# Autodesk Inventor assembly: клешня сбора
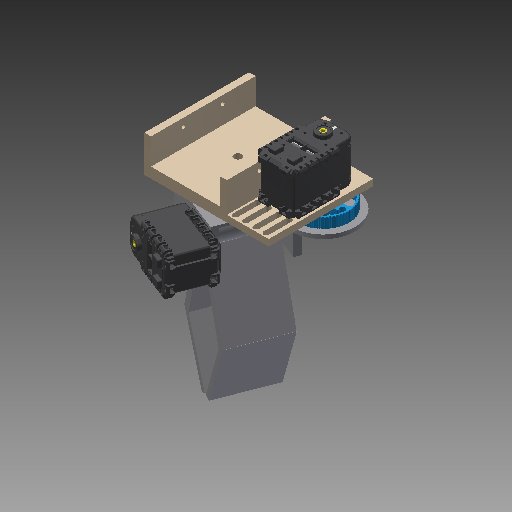
[picture p0: Inventor's stored thumbnail of the model, 512x512]
Saved by Autodesk Inventor 2019 (Build 230136000, 136)
## iProperties
Created: 2019-08-15
Part Number: клешня сбора
Material: Типовые
Document SubType Name: Assembly
Designer: Петров Иван
Author: Петров Иван
## Documents named in this file (8)
- C:\Users\user\Documents\Kvantoriada2019\optimal_gripper\hardware\Стандартные изделия\Концевик механический\клешня\клешня сбора.iam
- C:\Users\user\Documents\Kvantoriada2019\optimal_gripper\hardware\КВ33.044.101 - Опора захвата.ipt
- C:\Users\user\Documents\Kvantoriada2019\optimal_gripper\hardware\Стандартные изделия\Сервомотор Dynamixel AX-12A\ax-12a.iam
- C:\Users\user\Documents\Kvantoriada2019\optimal_gripper\hardware\Стандартные изделия\Проставка 4 мм.ipt
- C:\Users\user\Documents\Kvantoriada2019\optimal_gripper\hardware\Стандартные изделия\Шкив большой Makeblock.ipt
- C:\Users\user\Documents\Kvantoriada2019\optimal_gripper\hardware\Стандартные изделия\Боковина шкива уменьшанная.ipt
- C:\Users\user\Documents\Kvantoriada2019\optimal_gripper\hardware\Стандартные изделия\Концевик механический\клешня\Шкив большой сборка.iam
- C:\Users\user\Documents\Kvantoriada2019\optimal_gripper\hardware\Стандартные изделия\Концевик механический\клешня\сборка захвата.iam
## Components (8 placed, 7 different names)
1. КВ33.044.101 - Опора захвата:1 — Совмещение:1, Совмещение:2, Совмещение:3, Совмещение:17, Совмещение:18
2. ax-12a:1 [sub-assembly] — Совмещение:1, Совмещение:2, Совмещение:3, Совмещение:4, Совмещение:5
3. Проставка 4 мм:1 — Совмещение:4, Совмещение:5, Совмещение:6, Совмещение:7, Совмещение:8
4. Шкив большой Makeblock:1 — Совмещение:6, Совмещение:7, Совмещение:8, Совмещение:14, Совмещение:15, Совмещение:16, Направление навивки:1
5. Боковина шкива уменьшанная:1 — Совмещение:14, Совмещение:15, Совмещение:16
6. Шкив большой сборка:1 [sub-assembly] — Совмещение:17, Совмещение:18, Направление навивки:1, Совмещение:19, Совмещение:20, Совмещение:21
7. Боковина шкива уменьшанная:2 — Совмещение:19, Совмещение:20, Совмещение:21, Совмещение:22, Совмещение:23, Совмещение:24
8. сборка захвата:1 [sub-assembly] — Совмещение:22, Совмещение:23, Совмещение:24
## Relationships (20: Mate 19, RelateRotation 1)
- Совмещение:1 [Mate]: КВ33.044.101 - Опора захвата:1 ↔ ax-12a:1
- Совмещение:2 [Mate]: КВ33.044.101 - Опора захвата:1 ↔ ax-12a:1
- Совмещение:3 [Mate]: КВ33.044.101 - Опора захвата:1 ↔ ax-12a:1
- Совмещение:4 [Mate]: ax-12a:1 ↔ Проставка 4 мм:1
- Совмещение:5 [Mate]: ax-12a:1 ↔ Проставка 4 мм:1
- Совмещение:6 [Mate]: Проставка 4 мм:1 ↔ Шкив большой Makeblock:1
- Совмещение:7 [Mate]: Проставка 4 мм:1 ↔ Шкив большой Makeblock:1
- Совмещение:8 [Mate]: Проставка 4 мм:1 ↔ Шкив большой Makeblock:1
- Совмещение:14 [Mate]: Шкив большой Makeblock:1 ↔ Боковина шкива уменьшанная:1
- Совмещение:15 [Mate]: Шкив большой Makeblock:1 ↔ Боковина шкива уменьшанная:1
- Совмещение:16 [Mate]: Шкив большой Makeblock:1 ↔ Боковина шкива уменьшанная:1
- Совмещение:17 [Mate] (4.24 mm): КВ33.044.101 - Опора захвата:1 ↔ Шкив большой сборка:1
- Совмещение:18 [Mate]: КВ33.044.101 - Опора захвата:1 ↔ Шкив большой сборка:1
- Направление навивки:1 [RelateRotation] (1 ul): Шкив большой Makeblock:1 ↔ Шкив большой сборка:1
- Совмещение:19 [Mate]: Шкив большой сборка:1 ↔ Боковина шкива уменьшанная:2
- Совмещение:20 [Mate]: Шкив большой сборка:1 ↔ Боковина шкива уменьшанная:2
- Совмещение:21 [Mate]: Шкив большой сборка:1 ↔ Боковина шкива уменьшанная:2
- Совмещение:22 [Mate]: Боковина шкива уменьшанная:2 ↔ сборка захвата:1
- Совмещение:23 [Mate]: Боковина шкива уменьшанная:2 ↔ сборка захвата:1
- Совмещение:24 [Mate]: Боковина шкива уменьшанная:2 ↔ сборка захвата:1
